# Autodesk Inventor assembly: ForeArm
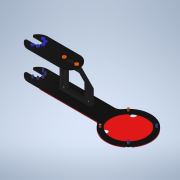
[picture p0: Inventor's stored thumbnail of the model, 180x180]
Saved by Autodesk Inventor 2020 (Build 240168000, 168)
## iProperties
Created: 2022-01-10
Part Number: ForeArm
Document SubType Name: Assembly
Designer: Masato Kubotera
Author: Masato Kubotera
## Documents named in this file (10)
- C:\Users\MasatoKubotera\Documents\Inventor\SUSTAINA-OP\UpperBody\Arm\ForeArm.iam
- C:\Users\MasatoKubotera\Documents\Inventor\SUSTAINA-OP\UpperBody\Arm\ForeArm_outside_frame.ipt
- C:\Users\MasatoKubotera\Documents\Inventor\SUSTAINA-OP\UpperBody\Arm\ForeArm_inside_frame.ipt
- C:\Users\MasatoKubotera\Documents\Inventor\SUSTAINA-OP\ReadyMade\Screw\M3-6.ipt
- C:\Users\MasatoKubotera\Documents\Inventor\SUSTAINA-OP\ReadyMade\Screw\M2_6-6.ipt
- C:\Users\MasatoKubotera\Documents\Inventor\SUSTAINA-OP\ReadyMade\InsertNut\IRU-304S.ipt
- C:\Users\MasatoKubotera\Documents\Inventor\SUSTAINA-OP\UpperBody\Arm\ForeArm_diagonal.ipt
- C:\Users\MasatoKubotera\Documents\Inventor\SUSTAINA-OP\UpperBody\Arm\ForeArm_outside_cloth.ipt
- C:\Users\MasatoKubotera\Documents\Inventor\SUSTAINA-OP\ReadyMade\Bush\L3040-8110TB.ipt
- C:\Users\MasatoKubotera\Documents\Inventor\SUSTAINA-OP\ReadyMade\Screw\M3-8.ipt
## Components (29 placed, 9 different names)
1. ForeArm_outside_frame:1 — 挿入:16, 挿入:17, 挿入:23, 挿入:24, 挿入:28, 挿入:31, 挿入:32, 挿入:33, 挿入:34, メイト:1, メイト:2, フラッシュ:1, 挿入:39, 挿入:41, 挿入:42, 挿入:43
2. ForeArm_inside_frame:1 — 挿入:25, 挿入:26, 挿入:29, 挿入:30, 挿入:35, 挿入:36, 挿入:37, 挿入:38, 挿入:40
3. ForeArm_diagonal:1 — 挿入:19, 挿入:20, 挿入:21, 挿入:22
4. M2_6-6:9 — 挿入:39
5. M2_6-6:10 — 挿入:40
6. ForeArm_outside_cloth:1 — 挿入:47, 挿入:48, 挿入:49
7. L3040-8110TB:1 — 挿入:41, 挿入:47, 挿入:50
8. L3040-8110TB:2 — 挿入:42, 挿入:48, 挿入:51
9. L3040-8110TB:3 — 挿入:43, 挿入:46, 挿入:49
10. M3-8:2 — 挿入:50
11. M3-8:3 — 挿入:51
12. M3-6:10 — 挿入:30
13. M3-6:9 — 挿入:29
14. M3-6:8 — 挿入:28
15. M2_6-6:8 — 挿入:38
16. M2_6-6:7 — 挿入:37
17. M2_6-6:6 — 挿入:36
18. M2_6-6:5 — 挿入:35
19. M2_6-6:4 — 挿入:34
20. M2_6-6:3 — 挿入:33
21. M2_6-6:2 — 挿入:32
22. M2_6-6:1 — 挿入:31
23. M3-6:5 — 挿入:17
24. M3-6:4 — 挿入:16
25. M3-8:1 — 挿入:46
26. IRU-304S:1 — 挿入:19, 挿入:23
27. IRU-304S:2 — 挿入:20, 挿入:24
28. IRU-304S:3 — 挿入:21, 挿入:25
29. IRU-304S:4 — 挿入:22, 挿入:26
## Relationships (35: Insert 32, Mate 2, Flush 1)
- 挿入:16 [Insert]: ForeArm_outside_frame:1 ↔ M3-6:4
- 挿入:17 [Insert]: ForeArm_outside_frame:1 ↔ M3-6:5
- 挿入:19 [Insert]: ForeArm_diagonal:1 ↔ IRU-304S:1
- 挿入:20 [Insert]: ForeArm_diagonal:1 ↔ IRU-304S:2
- 挿入:21 [Insert]: ForeArm_diagonal:1 ↔ IRU-304S:3
- 挿入:22 [Insert]: ForeArm_diagonal:1 ↔ IRU-304S:4
- 挿入:23 [Insert]: ForeArm_outside_frame:1 ↔ IRU-304S:1
- 挿入:24 [Insert]: ForeArm_outside_frame:1 ↔ IRU-304S:2
- 挿入:25 [Insert]: ForeArm_inside_frame:1 ↔ IRU-304S:3
- 挿入:26 [Insert]: ForeArm_inside_frame:1 ↔ IRU-304S:4
- 挿入:28 [Insert]: ForeArm_outside_frame:1 ↔ M3-6:8
- 挿入:29 [Insert]: ForeArm_inside_frame:1 ↔ M3-6:9
- 挿入:30 [Insert]: ForeArm_inside_frame:1 ↔ M3-6:10
- 挿入:31 [Insert]: ForeArm_outside_frame:1 ↔ M2_6-6:1
- 挿入:32 [Insert]: ForeArm_outside_frame:1 ↔ M2_6-6:2
- 挿入:33 [Insert]: ForeArm_outside_frame:1 ↔ M2_6-6:3
- 挿入:34 [Insert]: ForeArm_outside_frame:1 ↔ M2_6-6:4
- 挿入:35 [Insert]: ForeArm_inside_frame:1 ↔ M2_6-6:5
- 挿入:36 [Insert]: ForeArm_inside_frame:1 ↔ M2_6-6:6
- 挿入:37 [Insert]: ForeArm_inside_frame:1 ↔ M2_6-6:7
- 挿入:38 [Insert]: ForeArm_inside_frame:1 ↔ M2_6-6:8
- メイト:1 [Mate]: ForeArm_outside_frame:1
- メイト:2 [Mate]: ForeArm_outside_frame:1
- フラッシュ:1 [Flush]: ForeArm_outside_frame:1
- 挿入:39 [Insert]: ForeArm_outside_frame:1 ↔ M2_6-6:9
- 挿入:40 [Insert]: ForeArm_inside_frame:1 ↔ M2_6-6:10
- 挿入:41 [Insert]: ForeArm_outside_frame:1 ↔ L3040-8110TB:1
- 挿入:42 [Insert]: ForeArm_outside_frame:1 ↔ L3040-8110TB:2
- 挿入:43 [Insert]: ForeArm_outside_frame:1 ↔ L3040-8110TB:3
- 挿入:46 [Insert]: L3040-8110TB:3 ↔ M3-8:1
- 挿入:47 [Insert]: ForeArm_outside_cloth:1 ↔ L3040-8110TB:1
- 挿入:48 [Insert]: ForeArm_outside_cloth:1 ↔ L3040-8110TB:2
- 挿入:49 [Insert]: ForeArm_outside_cloth:1 ↔ L3040-8110TB:3
- 挿入:50 [Insert]: L3040-8110TB:1 ↔ M3-8:2
- 挿入:51 [Insert]: L3040-8110TB:2 ↔ M3-8:3
